# Autodesk Inventor assembly: Assembly
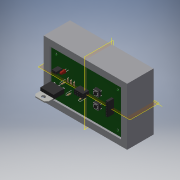
[picture p0: Inventor's stored thumbnail of the model, 180x180]
Saved by Autodesk Inventor 2018 (Build 220112000, 112)
## iProperties
Created: 2018-09-30
Part Number: Assembly
Document SubType Name: Assembly
Designer: andfro
Author: andfro
## iProperties of the stored document PinSocket_1x02_P2.54mm_Vertical.iam
Created: 2018-09-30
Part Number: PinSocket_1x02_P2.54mm_Vertical
Document SubType Name: Assembly
Designer: andfro
Author: andfro
## iProperties of the stored document PinSocket_1x06_P2.54mm_Vertical.iam
Created: 2018-09-30
Part Number: PinSocket_1x06_P2.54mm_Vertical
Document SubType Name: Assembly
Designer: andfro
Author: andfro
## iProperties of the stored document R_Axial_DIN0204_L3.6mm_D1.6mm_P5.08mm_Horizontal.iam
Created: 2018-09-30
Part Number: R_Axial_DIN0204_L3.6mm_D1.6mm_P5.08mm_Horizontal
Document SubType Name: Assembly
Designer: andfro
Author: andfro
## iProperties of the stored document SOLID_5.ipt
Created: 2018-09-30
Part Number: SOLID_5
Material: Generic
Document SubType Name: Modeling
Designer: andfro
Density: 1 g/cm^3
Appearance: Default
Author: andfro
## iProperties of the stored document SOLID_2.ipt
Created: 2018-09-30
Part Number: SOLID_2
Material: Generic
Document SubType Name: Modeling
Designer: andfro
Density: 1 g/cm^3
Appearance: Default
Author: andfro
## iProperties of the stored document SOLID_3.ipt
Created: 2018-09-30
Part Number: SOLID_3
Material: Generic
Document SubType Name: Modeling
Designer: andfro
Density: 1 g/cm^3
Appearance: Default
Author: andfro
## iProperties of the stored document SW_PUSH_6mm_H4.3mm.iam
Created: 2018-09-30
Part Number: SW_PUSH_6mm_H4.3mm
Document SubType Name: Assembly
Designer: andfro
Author: andfro
## iProperties of the stored document LED_D3.0mm.iam
Created: 2018-09-30
Part Number: LED_D3.0mm
Document SubType Name: Assembly
Designer: andfro
Author: andfro
## iProperties of the stored document PinSocket_2x04_P2.54mm_Vertical.iam
Created: 2018-09-30
Part Number: PinSocket_2x04_P2.54mm_Vertical
Document SubType Name: Assembly
Designer: andfro
Author: andfro
## iProperties of the stored document TO-218-3_Vertical.iam
Created: 2018-09-30
Part Number: TO-218-3_Vertical
Document SubType Name: Assembly
Designer: andfro
Author: andfro
## iProperties of the stored document SOLID.ipt
Created: 2018-09-30
Part Number: SOLID
Material: Generic
Document SubType Name: Modeling
Designer: andfro
Density: 1 g/cm^3
Appearance: Default
Author: andfro
## iProperties of the stored document SOLID_8.ipt
Created: 2018-09-30
Part Number: SOLID_8
Material: Generic
Document SubType Name: Modeling
Designer: andfro
Density: 1 g/cm^3
Appearance: Default
Author: andfro
## iProperties of the stored document SOLID_6.ipt
Created: 2018-09-30
Part Number: SOLID_6
Material: Generic
Document SubType Name: Modeling
Designer: andfro
Density: 1 g/cm^3
Appearance: Default
Author: andfro
## iProperties of the stored document SOLID_4.ipt
Created: 2018-09-30
Part Number: SOLID_4
Material: Generic
Document SubType Name: Modeling
Designer: andfro
Density: 1 g/cm^3
Appearance: Default
Author: andfro
## iProperties of the stored document SOLID_1.ipt
Created: 2018-09-30
Part Number: SOLID_1
Material: Generic
Document SubType Name: Modeling
Designer: andfro
Density: 1 g/cm^3
Appearance: Default
Author: andfro
## iProperties of the stored document SOLID_7.ipt
Created: 2018-09-30
Part Number: SOLID_7
Material: Generic
Document SubType Name: Modeling
Designer: andfro
Density: 1 g/cm^3
Appearance: Default
Author: andfro
## iProperties of the stored document C_0805_2012Metric.iam
Created: 2018-09-30
Part Number: C_0805_2012Metric
Document SubType Name: Assembly
Designer: andfro
Author: andfro
## iProperties of the stored document R_Axial_DIN0204_L3.6mm_D1.6mm_P2.54mm_Vertical.iam
Created: 2018-09-30
Part Number: R_Axial_DIN0204_L3.6mm_D1.6mm_P2.54mm_Vertical
Document SubType Name: Assembly
Designer: andfro
Author: andfro
## iProperties of the stored document COMPOUND.ipt
Created: 2018-09-30
Part Number: COMPOUND
Material: Generic
Document SubType Name: Modeling
Designer: andfro
Density: 1 g/cm^3
Appearance: Default
Author: andfro
## iProperties of the stored document esp01_programmer.iam
Company: A Company
Created: 2018-09-30
Part Number: esp01_programmer
Description: KiCad electronic assembly
Document SubType Name: Assembly
Designer: andfro
Authority: Unknown
Title: esp01_programmer.step
Author: An Author
Sending System: KiCad to STEP converter
Preprocessor: Open CASCADE STEP processor 6.8
## Documents named in this file (23)
- C:\Users\andfro\Documents\Projects\esp01_programmer\MCAD\Assembly.iam
- C:\Users\andfro\Documents\Projects\esp01_programmer\MCAD\Case.ipt
- **C:\Users\andfro\Documents\Projects\esp01_programmer\MCAD\Assembly.iam*LocalDocs*xXogaobuw1cbguiw3Dl4v3x5oDe*esp01_programmer.iam
- **C:\Users\andfro\Documents\Projects\esp01_programmer\MCAD\Assembly.iam*LocalDocs*xFdj1yqyqHfz4uko0I0u2inraPh*PinSocket_1x02_P2.54mm_Vertical.iam
- **C:\Users\andfro\Documents\Projects\esp01_programmer\MCAD\Assembly.iam*LocalDocs*xFmlet5bgAxahedw12epn02eoUe*SOLID_8.ipt
- **C:\Users\andfro\Documents\Projects\esp01_programmer\MCAD\Assembly.iam*LocalDocs*xCr4g2b4cY4jsupky3swe2pe1Sg*PinSocket_1x06_P2.54mm_Vertical.iam
- **C:\Users\andfro\Documents\Projects\esp01_programmer\MCAD\Assembly.iam*LocalDocs*xGa1bexmjDamtuq04Ssyw42rkZf*SOLID_6.ipt
- **C:\Users\andfro\Documents\Projects\esp01_programmer\MCAD\Assembly.iam*LocalDocs*x5rzdatq0ZvzdepwyC554x3xfAe*R_Axial_DIN0204_L3.6mm_D1.6mm_P5.08mm_Horizontal.iam
- **C:\Users\andfro\Documents\Projects\esp01_programmer\MCAD\Assembly.iam*LocalDocs*xGqe1dpkaT151e0ojZtkzhwrrFh*SOLID.ipt
- **C:\Users\andfro\Documents\Projects\esp01_programmer\MCAD\Assembly.iam*LocalDocs*x3udh1qf4214bud45F4ogdgvc5b*SOLID_5.ipt
- **C:\Users\andfro\Documents\Projects\esp01_programmer\MCAD\Assembly.iam*LocalDocs*x2ssw0lvzEzy2ersyMg5xzyr4Th*SOLID_2.ipt
- **C:\Users\andfro\Documents\Projects\esp01_programmer\MCAD\Assembly.iam*LocalDocs*xBbanbhs2ZedxedslWcnwn40eSh*SOLID_3.ipt
- **C:\Users\andfro\Documents\Projects\esp01_programmer\MCAD\Assembly.iam*LocalDocs*xE4iibzg0N2aauhwlZsnd1ffdDd*SW_PUSH_6mm_H4.3mm.iam
- **C:\Users\andfro\Documents\Projects\esp01_programmer\MCAD\Assembly.iam*LocalDocs*xLfg3n3dsHcaou0klCadtrckwQc*SOLID_7.ipt
- **C:\Users\andfro\Documents\Projects\esp01_programmer\MCAD\Assembly.iam*LocalDocs*xDajssx5y5otjuo03S4fht45kLa*LED_D3.0mm.iam
- **C:\Users\andfro\Documents\Projects\esp01_programmer\MCAD\Assembly.iam*LocalDocs*xEwygzs3e0bsqexofE4oxcfplHf*PinSocket_2x04_P2.54mm_Vertical.iam
- **C:\Users\andfro\Documents\Projects\esp01_programmer\MCAD\Assembly.iam*LocalDocs*xK05grzxjMirdussiGfhrp3ykRh*SOLID_1.ipt
- **C:\Users\andfro\Documents\Projects\esp01_programmer\MCAD\Assembly.iam*LocalDocs*xNv0re551Izf4u1ghOxvkgujvPc*TO-218-3_Vertical.iam
- **C:\Users\andfro\Documents\Projects\esp01_programmer\MCAD\Assembly.iam*LocalDocs*xKgogij51R2pwu5w0Mdzda2rb3g*SOLID_4.ipt
- **C:\Users\andfro\Documents\Projects\esp01_programmer\MCAD\Assembly.iam*LocalDocs*xVnax3d3lJeyauh445a3hlfvwAg*C_0805_2012Metric.iam
- **C:\Users\andfro\Documents\Projects\esp01_programmer\MCAD\Assembly.iam*LocalDocs*xTk5evaosJh2tuewe3v5wum4q3h*R_Axial_DIN0204_L3.6mm_D1.6mm_P2.54mm_Vertical.iam
- **C:\Users\andfro\Documents\Projects\esp01_programmer\MCAD\Assembly.iam*LocalDocs*xXf53bk0xOzfwe30e32kvcz5q0f*COMPOUND.ipt
- C:\Users\andfro\Documents\Projects\esp01_programmer\esp01_programmer.step
## Components (2 placed, 2 different names)
1. Case:1 — Mate:2, Mate:3, Mate:4
2. esp01_programmer:1 [sub-assembly] — Mate:2, Mate:3, Mate:4
## Relationships (3: Mate 3)
- Mate:2: Case:1 ↔ esp01_programmer:1
- Mate:3: Case:1 ↔ esp01_programmer:1
- Mate:4: Case:1 ↔ esp01_programmer:1
